# Autodesk Inventor assembly: CAD_1
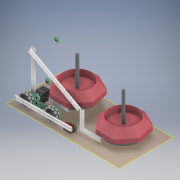
[picture p0: Inventor's stored thumbnail of the model, 180x180]
Saved by Autodesk Inventor 2022 (Build 260153000, 153)
## iProperties
Created: 2021-05-23
Part Number: CAD_1
Document SubType Name: Assembly
Designer: carlo
Author: carlo
## Documents named in this file (13)
- C:\the7dorks.github.io\CAD_1.iam
- C:\the7dorks.github.io\Library 1.2\Motion\Wheels\Omnis\4 Omni, Square.ipt
- C:\the7dorks.github.io\Library 1.2\Structure\C-Channels\Aluminum 1x2x1\1x2x1x35 Aluminum.ipt
- C:\the7dorks.github.io\Library 1.2\Motion\Gears\HS 84T Gear, Square.ipt
- C:\the7dorks.github.io\Library 1.2\Motion\Gears\HS 36T Gear, Square.ipt
- C:\the7dorks.github.io\Library 1.2\Motion\Gears\HS 36T Gear, Circle.ipt
- C:\the7dorks.github.io\Library 1.2\Electronics\Sensors\Optical Shaft Encoder.ipt
- C:\the7dorks.github.io\Library 1.2\Motion\Wheels\Omnis\2.75 Omni - Old.ipt
- C:\the7dorks.github.io\Library 1.2\Electronics\V5 Motor.ipt
- C:\the7dorks.github.io\Tipping Poing Field CAD\Alliance_Mobile_Goal_Red.iam
- C:\the7dorks.github.io\Library 1.2\Structure\C-Channels\Aluminum 1x2x1\1x2x1x12 Aluminum.ipt
- C:\the7dorks.github.io\Library 1.2\Structure\C-Channels\Aluminum 1x2x1\1x2x1x25 Aluminum.ipt
- C:\the7dorks.github.io\Library 1.2\Motion\Sprockets\HS 12T Sprocket, Square.ipt
## Components (22 placed, 12 different names)
1. 1x2x1x35 Aluminum:1 — Flush:7, Mate:1, Mate:2
2. 4 Omni, Square:1
3. HS 84T Gear, Square:1
4. HS 36T Gear, Square:1
5. 4 Omni, Square:2
6. HS 84T Gear, Square:2
7. HS 36T Gear, Square:2
8. HS 36T Gear, Circle:1
9. HS 36T Gear, Circle:2
10. 2.75 Omni - Old:1
11. Optical Shaft Encoder:1
12. V5 Motor:1
13. V5 Motor:2
14. Alliance_Mobile_Goal_Red:1 [sub-assembly]
15. 1x2x1x12 Aluminum:1
16. 1x2x1x25 Aluminum:1
17. 1x2x1x35 Aluminum:2
18. Alliance_Mobile_Goal_Red:2 [sub-assembly]
19. 1x2x1x12 Aluminum:2
20. 1x2x1x12 Aluminum:3
21. HS 12T Sprocket, Square:1
22. HS 12T Sprocket, Square:2
## Relationships (9: Flush 7, Mate 2)
- Flush:1 (228.6 mm)
- Flush:2 (-228.6 mm)
- Flush:3 (228.6 mm)
- Flush:4 (-228.6 mm)
- Flush:5 (457.2 mm)
- Flush:6
- Flush:7: 1x2x1x35 Aluminum:1
- Mate:1: 1x2x1x35 Aluminum:1
- Mate:2 (40.386 mm): 1x2x1x35 Aluminum:1
